# Autodesk Inventor assembly: Robotic Arm Assembly 1(new)
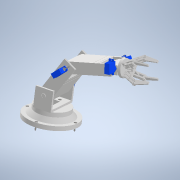
[picture p0: Inventor's stored thumbnail of the model, 180x180]
Saved by Autodesk Inventor 2022 (Build 260153000, 153)
## iProperties
Created: 2021-07-27
Part Number: Robotic Arm Assembly 1(new)
Document SubType Name: Assembly
Designer: USER
Author: USER
## Documents named in this file (17)
- F:\BVB\robotic arm\Robotic Arm Assembly 1(new).iam
- F:\BVB\robotic arm\base 1.ipt
- F:\BVB\robotic arm\1st arm.ipt
- F:\BVB\robotic arm\1st arm closing.ipt
- F:\BVB\robotic arm\1st arm and clamp pin.ipt
- F:\BVB\robotic arm\base 1st arm pin.ipt
- F:\BVB\robotic arm\base and 1st arm link.ipt
- F:\BVB\robotic arm\screw EE.ipt
- F:\BVB\robotic arm\1st arm to 2nd linking clamp.ipt
- F:\BVB\robotic arm\2nd arm.ipt
- F:\BVB\robotic arm\2nd arm closing.ipt
- F:\BVB\robotic arm\2nd arm and clamp pin.ipt
- F:\BVB\robotic arm\2nd to 3rd arm linking clamp.ipt
- F:\BVB\robotic arm\3rd arm.ipt
- F:\BVB\robotic arm\3rd arm motor pin.ipt
- F:\BVB\robotic arm\Servo Motor SG90.ipt
- F:\BVB\robotic arm\gripper assembly 1.iam
## Components (35 placed, 16 different names)
1. base 1:1 — Mate:5, Flush:5, Flush:6, Mate:37, Mate:38, Mate:39, Mate:40, Flush:26, Flush:27, Flush:28, Flush:29
2. 1st arm:1 — Mate:2, Flush:3, Flush:4, Mate:7, Rotational:4
3. 1st arm closing:1 — Mate:2, Flush:3, Flush:4, Mate:10, Flush:9, Flush:10
4. base 1st arm pin:1 — Mate:6, Rotational:1, Mate:30, Mate:31
5. base and 1st arm link:1 — Mate:5, Flush:5, Flush:6, Mate:6, Rotational:1, Mate:7, Mate:8, Flush:7, Mate:9, Flush:8, Rotational:4
6. screw EE:1 — Mate:8, Flush:7
7. screw EE:2 — Mate:9, Flush:8
8. screw EE:3 — Mate:11, Flush:12
9. screw EE:4 — Mate:18, Flush:17
10. screw EE:5 — Mate:25, Flush:19
11. screw EE:6 — Mate:24, Flush:20
12. screw EE:7 — Mate:29, Flush:21
13. screw EE:8 — Mate:28, Flush:22
14. screw EE:9 — Mate:17, Flush:18
15. screw EE:10 — Mate:12, Flush:11
16. 1st arm to 2nd linking clamp:1 — Mate:10, Flush:9, Flush:10, Mate:11, Mate:12, Flush:11, Flush:12, Mate:14, Rotational:3, Rotational:5
17. 1st arm and clamp pin:1 — Mate:14, Rotational:3, Mate:15, Mate:26, Mate:27
18. 2nd arm:1 — Mate:13, Flush:13, Flush:14, Mate:15, Rotational:5, Flush:15
19. 2nd arm closing:1 — Mate:13, Flush:13, Flush:14, Mate:16, Flush:16
20. 2nd arm and clamp pin:1 — Mate:19, Rotational:6, Mate:20, Mate:23
21. 2nd to 3rd arm linking clamp:1 — Mate:16, Flush:15, Flush:16, Mate:17, Mate:18, Flush:17, Flush:18, Mate:19, Rotational:6, Rotational:7, Mate:22
22. 3rd arm:1 — Mate:20, Rotational:7, Mate:21, Rotational:8, Mate:41, Mate:42, Mate:43
23. 3rd arm motor pin:1 — Mate:21, Rotational:8, Mate:34, Mate:35
24. Servo Motor SG90:1 — Mate:22, Mate:23, Mate:24, Mate:25, Flush:19, Flush:20
25. Servo Motor SG90:2 — Mate:26, Mate:27, Mate:28, Mate:29, Flush:21, Flush:22
26. Servo Motor SG90:3 — Mate:34, Mate:35, Mate:36, Flush:25
27. Servo Motor SG90:4 — Mate:30, Mate:31, Mate:32, Mate:33, Flush:23, Flush:24
28. screw EE:11 — Mate:32, Flush:24
29. screw EE:13 — Mate:36, Flush:25
30. screw EE:14 — Mate:33, Flush:23
31. screw EE:15 — Mate:40, Flush:26
32. screw EE:16 — Mate:38, Flush:27
33. screw EE:17 — Mate:37, Flush:28
34. screw EE:18 — Mate:39, Flush:29
35. gripper assembly 1:1 [sub-assembly] — Mate:41, Mate:42, Mate:43
## Relationships (74: Mate 40, Flush 27, RevoluteJoint 7)
- Mate:2: 1st arm:1 ↔ 1st arm closing:1
- Flush:3: 1st arm:1 ↔ 1st arm closing:1
- Flush:4: 1st arm:1 ↔ 1st arm closing:1
- Mate:5: base 1:1 ↔ base and 1st arm link:1
- Flush:5 (1 mm): base 1:1 ↔ base and 1st arm link:1
- Flush:6: base 1:1 ↔ base and 1st arm link:1
- Mate:6: base 1st arm pin:1 ↔ base and 1st arm link:1
- Rotational:1 [RevoluteJoint]: base 1st arm pin:1 ↔ base and 1st arm link:1
- Mate:7 (1 mm): 1st arm:1 ↔ base and 1st arm link:1
- Mate:8: base and 1st arm link:1 ↔ screw EE:1
- Flush:7: base and 1st arm link:1 ↔ screw EE:1
- Mate:9: base and 1st arm link:1 ↔ screw EE:2
- Flush:8: base and 1st arm link:1 ↔ screw EE:2
- Mate:10: 1st arm closing:1 ↔ 1st arm to 2nd linking clamp:1
- Flush:9: 1st arm closing:1 ↔ 1st arm to 2nd linking clamp:1
- Flush:10: 1st arm closing:1 ↔ 1st arm to 2nd linking clamp:1
- Mate:11: screw EE:3 ↔ 1st arm to 2nd linking clamp:1
- Mate:12: screw EE:10 ↔ 1st arm to 2nd linking clamp:1
- Flush:11: screw EE:10 ↔ 1st arm to 2nd linking clamp:1
- Flush:12: screw EE:3 ↔ 1st arm to 2nd linking clamp:1
- Mate:13: 2nd arm:1 ↔ 2nd arm closing:1
- Flush:13: 2nd arm:1 ↔ 2nd arm closing:1
- Flush:14: 2nd arm:1 ↔ 2nd arm closing:1
- Mate:14: 1st arm to 2nd linking clamp:1 ↔ 1st arm and clamp pin:1
- Rotational:3 [RevoluteJoint]: 1st arm to 2nd linking clamp:1 ↔ 1st arm and clamp pin:1
- Mate:15: 1st arm and clamp pin:1 ↔ 2nd arm:1
- Rotational:4 [RevoluteJoint] (1 mm): 1st arm:1 ↔ base and 1st arm link:1
- Rotational:5 [RevoluteJoint] (-1.5 mm): 1st arm to 2nd linking clamp:1 ↔ 2nd arm:1
- Mate:16: 2nd arm closing:1 ↔ 2nd to 3rd arm linking clamp:1
- Flush:15: 2nd arm:1 ↔ 2nd to 3rd arm linking clamp:1
- Flush:16: 2nd arm closing:1 ↔ 2nd to 3rd arm linking clamp:1
- Mate:17: screw EE:9 ↔ 2nd to 3rd arm linking clamp:1
- Mate:18: screw EE:4 ↔ 2nd to 3rd arm linking clamp:1
- Flush:17: screw EE:4 ↔ 2nd to 3rd arm linking clamp:1
- Flush:18: screw EE:9 ↔ 2nd to 3rd arm linking clamp:1
- Mate:19: 2nd arm and clamp pin:1 ↔ 2nd to 3rd arm linking clamp:1
- Rotational:6 [RevoluteJoint]: 2nd arm and clamp pin:1 ↔ 2nd to 3rd arm linking clamp:1
- Mate:20: 2nd arm and clamp pin:1 ↔ 3rd arm:1
- Rotational:7 [RevoluteJoint] (2.5 mm): 2nd to 3rd arm linking clamp:1 ↔ 3rd arm:1
- Mate:21: 3rd arm:1 ↔ 3rd arm motor pin:1
- Rotational:8 [RevoluteJoint]: 3rd arm:1 ↔ 3rd arm motor pin:1
- Mate:22: 2nd to 3rd arm linking clamp:1 ↔ Servo Motor SG90:1
- Mate:23: 2nd arm and clamp pin:1 ↔ Servo Motor SG90:1
- Mate:24: screw EE:6 ↔ Servo Motor SG90:1
- Mate:25: screw EE:5 ↔ Servo Motor SG90:1
- Flush:19 (-3 mm): screw EE:5 ↔ Servo Motor SG90:1
- Flush:20 (-3 mm): screw EE:6 ↔ Servo Motor SG90:1
- Mate:26: 1st arm and clamp pin:1 ↔ Servo Motor SG90:2
- Mate:27: 1st arm and clamp pin:1 ↔ Servo Motor SG90:2
- Mate:28: screw EE:8 ↔ Servo Motor SG90:2
- Mate:29: screw EE:7 ↔ Servo Motor SG90:2
- Flush:21 (-3 mm): screw EE:7 ↔ Servo Motor SG90:2
- Flush:22 (-3 mm): screw EE:8 ↔ Servo Motor SG90:2
- Mate:30: base 1st arm pin:1 ↔ Servo Motor SG90:4
- Mate:31: base 1st arm pin:1 ↔ Servo Motor SG90:4
- Mate:32: Servo Motor SG90:4 ↔ screw EE:11
- Mate:33: Servo Motor SG90:4 ↔ screw EE:14
- Flush:23 (-3 mm): Servo Motor SG90:4 ↔ screw EE:14
- Flush:24 (3 mm): Servo Motor SG90:4 ↔ screw EE:11
- Mate:34: 3rd arm motor pin:1 ↔ Servo Motor SG90:3
- Mate:35: 3rd arm motor pin:1 ↔ Servo Motor SG90:3
- Mate:36: Servo Motor SG90:3 ↔ screw EE:13
- Flush:25 (-3 mm): Servo Motor SG90:3 ↔ screw EE:13
- Mate:37: base 1:1 ↔ screw EE:17
- Mate:38: base 1:1 ↔ screw EE:16
- Mate:39: base 1:1 ↔ screw EE:18
- Mate:40: base 1:1 ↔ screw EE:15
- Flush:26: base 1:1 ↔ screw EE:15
- Flush:27: base 1:1 ↔ screw EE:16
- Flush:28: base 1:1 ↔ screw EE:17
- Flush:29: base 1:1 ↔ screw EE:18
- Mate:41: 3rd arm:1 ↔ gripper assembly 1:1
- Mate:42 (-10 mm): 3rd arm:1 ↔ gripper assembly 1:1
- Mate:43 (-20 mm): 3rd arm:1 ↔ gripper assembly 1:1
